# Autodesk Inventor assembly: Red Alliance Bucket
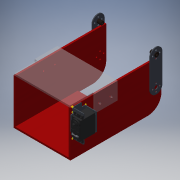
[picture p0: Inventor's stored thumbnail of the model, 180x180]
Saved by Autodesk Inventor 2016 (Build 200138000, 138)
## iProperties
Created: 2015-12-17
Part Number: Red Alliance Bucket
Document SubType Name: Assembly
Designer: TimB
Author: TimB
## Documents named in this file (7)
- C:\Users\TimB\Documents\GitHub\phi_robotics\3d-models\FTC_Tetrix_KOP_Block_Party\Tim Bloot Designs\JAr JaR Bot\Red Alliance Bucket.iam
- C:\Users\TimB\Documents\GitHub\phi_robotics\3d-models\FTC_Tetrix_KOP_Block_Party\Tim Bloot Designs\JAr JaR Bot\Bucket - RedA.ipt
- C:\Users\TimB\Documents\GitHub\phi_robotics\3d-models\FTC_Tetrix_KOP_Block_Party\Tetrix_Kit_FTC\Autodesk Inventor Files\tetrix_739061_2012.ipt
- C:\Users\TimB\Documents\GitHub\phi_robotics\3d-models\FTC_Tetrix_KOP_Block_Party\Tim Bloot Designs\JAr JaR Bot\Bucket -  Top.ipt
- C:\Users\TimB\Documents\GitHub\phi_robotics\3d-models\FTC_Tetrix_KOP_Block_Party\Tetrix_Kit_FTC\Autodesk Inventor Files\tetrix_servo_mount.ipt
- C:\Users\TimB\Documents\GitHub\phi_robotics\3d-models\FTC_Tetrix_KOP_Block_Party\Tetrix_Kit_FTC\Autodesk Inventor Files\tetrix_servo_body.ipt
- C:\Users\TimB\Documents\GitHub\phi_robotics\3d-models\FTC_Tetrix_KOP_Block_Party\Tetrix_Kit_FTC\Autodesk Inventor Files\tetrix_bushing.ipt
## Components (8 placed, 6 different names)
1. Bucket - RedA:1 — Rigid:1, Rigid:2, Rigid:3, Rigid:4
2. tetrix_739061_2012:1 — Rigid:1, Rotational:2
3. tetrix_739061_2012:2 — Rigid:2, Rotational:1
4. Bucket -  Top:1 — Rigid:3
5. tetrix_servo_mount:1 — Rigid:4, Rigid:5
6. tetrix_servo_body:1 — Rigid:5
7. tetrix_bushing:1 — Rotational:2
8. tetrix_bushing:2 — Rotational:1
## Relationships (7: WeldJoint 5, RevoluteJoint 2)
- Rigid:1 [WeldJoint]: Bucket - RedA:1 ↔ tetrix_739061_2012:1
- Rigid:2 [WeldJoint]: Bucket - RedA:1 ↔ tetrix_739061_2012:2
- Rigid:3 [WeldJoint]: Bucket - RedA:1 ↔ Bucket -  Top:1
- Rigid:4 [WeldJoint]: Bucket - RedA:1 ↔ tetrix_servo_mount:1
- Rigid:5 [WeldJoint]: tetrix_servo_mount:1 ↔ tetrix_servo_body:1
- Rotational:1 [RevoluteJoint]: tetrix_739061_2012:2 ↔ tetrix_bushing:2
- Rotational:2 [RevoluteJoint]: tetrix_739061_2012:1 ↔ tetrix_bushing:1
